# Autodesk Inventor assembly: 64아이들러
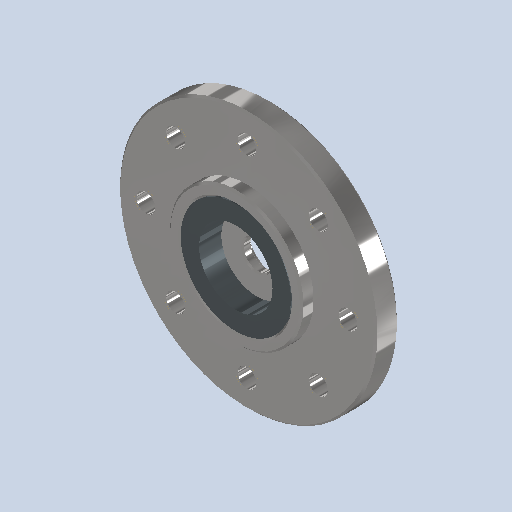
[picture p0: Inventor's stored thumbnail of the model, 512x512]
Saved by Autodesk Inventor 2024.3 (Build 283343000, 343)
## iProperties
Created: 2022-08-09
Part Number: 64아이들러
Document SubType Name: Assembly
Designer: 박지훈
Mass: 5 g
Surface Area: 21.0198 cm^2
Volume: 1.54681 cm^3
Author: 박지훈
## Documents named in this file (4)
- C:\Users\gretc\Desktop\inventor_part\아이들러\64아이들러.iam
- C:\Users\gretc\Desktop\inventor_part\아이들러\HN05-i1.ipt
- C:\Users\gretc\Desktop\inventor_part\아이들러\MF128ZZ.ipt
- C:\Users\gretc\Desktop\inventor_part\아이들러\RX64-CAP.ipt
## Components (3 placed, 3 different names)
1. HN05-i1:1 — 삽입:1
2. MF128ZZ:1 — 삽입:1, 삽입:2
3. RX64-CAP:1 — 삽입:2
## Relationships (2: Insert 2)
- 삽입:1 [Insert]: HN05-i1:1 ↔ MF128ZZ:1
- 삽입:2 [Insert]: MF128ZZ:1 ↔ RX64-CAP:1
